# Autodesk Inventor assembly: HP2 Raceparts Complette Tyre
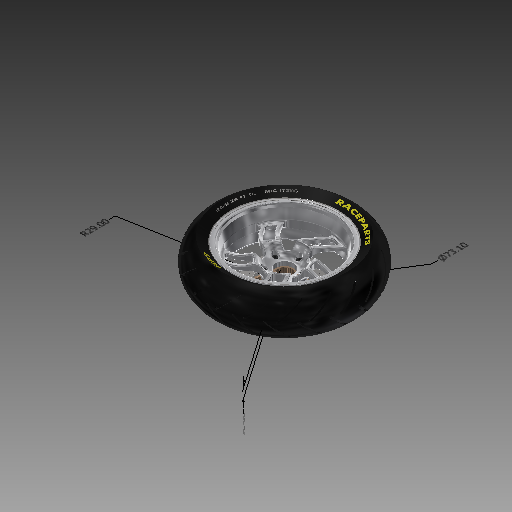
[picture p0: Inventor's stored thumbnail of the model, 512x512]
Saved by Autodesk Inventor 2019 (Build 230136000, 136)
## iProperties
Part Number: HP2 Raceparts Complette Tyre
Material: Generisch
Document SubType Name: Assembly
Designer: Catweazle
Author: Catweazle
## Documents named in this file (5)
- C:\Users\Administrator\Desktop\机械产品数字化设计大赛\轮腿\轮子\HP2 Raceparts Complette Tyre.iam
- C:\Users\Administrator\Desktop\机械产品数字化设计大赛\轮腿\轮子\HP2 Raceparts.iam
- C:\Users\Administrator\Desktop\机械产品数字化设计大赛\轮腿\轮子\HP2 Raceparts 003.ipt
- C:\Users\Administrator\Desktop\机械产品数字化设计大赛\轮腿\轮子\HP2 Raceparts 004.ipt
- C:\Users\Administrator\Desktop\机械产品数字化设计大赛\轮腿\轮子\HP2 Raceparts 005.ipt
## Components (8 placed, 4 different names)
1. HP2 Raceparts:1 [sub-assembly] — Passend:1, Passend:2, Passend:3
2. HP2 Raceparts 003:1 — Passend:1, Passend:2, Passend:3, Passend:4, Passend:5, Passend:6, Einfügen:1
3. HP2 Raceparts 004:1 — Passend:4, Passend:5
4. HP2 Raceparts 005:1 — Passend:6, Einfügen:1
5. HP2 Raceparts 005:2
6. HP2 Raceparts 005:3
7. HP2 Raceparts 005:4
8. HP2 Raceparts 005:5
## Component patterns: (5 elements, first: HP2 Raceparts 005:1)
## Relationships (7: Mate 6, Insert 1)
- Passend:1 [Mate]: HP2 Raceparts:1 ↔ HP2 Raceparts 003:1
- Passend:2 [Mate]: HP2 Raceparts:1 ↔ HP2 Raceparts 003:1
- Passend:3 [Mate]: HP2 Raceparts:1 ↔ HP2 Raceparts 003:1
- Passend:4 [Mate]: HP2 Raceparts 003:1 ↔ HP2 Raceparts 004:1
- Passend:5 [Mate]: HP2 Raceparts 003:1 ↔ HP2 Raceparts 004:1
- Passend:6 [Mate]: HP2 Raceparts 003:1 ↔ HP2 Raceparts 005:1
- Einfügen:1 [Insert]: HP2 Raceparts 003:1 ↔ HP2 Raceparts 005:1
